# Autodesk Inventor assembly: Motor
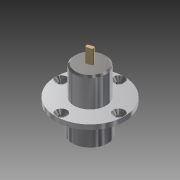
[picture p0: Inventor's stored thumbnail of the model, 180x180]
Saved by Autodesk Inventor 2014 SP1 (Build 180222100, 222)
## iProperties
Created: 2015-04-11
Part Number: Motor
Document SubType Name: Assembly
Designer: david
Mass: 73.49 g
Surface Area: 59.6795 cm^2
Volume: 16.2439 cm^3
Density: 4.52416 g/cm^3
Author: david
## Documents named in this file (3)
- C:\Users\asus\Documents\Autodesk\Projects\AUSBEEDone\Components\Motors\Motor.iam
- C:\Users\asus\Documents\Autodesk\Projects\AUSBEEDone\Components\Motors\MotorBody.ipt
- C:\Users\asus\Documents\Autodesk\Projects\AUSBEEDone\Components\Motors\MotorShaft.ipt
## Components (2 placed, 2 different names)
1. MotorBody:1 — Insert:1
2. MotorShaft:1 — Insert:1
## Relationships (1: Insert 1)
- Insert:1: MotorBody:1 ↔ MotorShaft:1
